# Autodesk Inventor assembly: MotorAndLoadCellBase
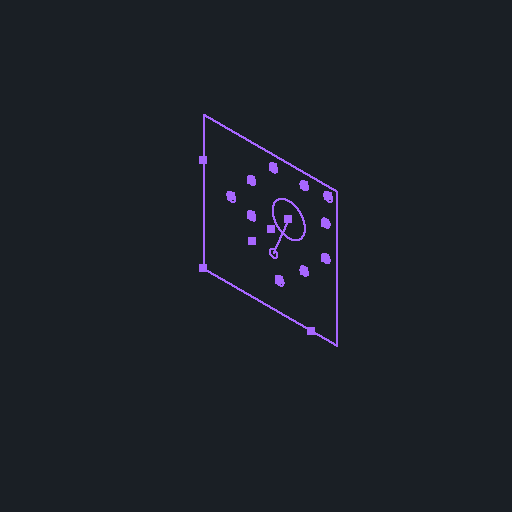
[picture p0: Inventor's stored thumbnail of the model, 512x512]
Saved by Autodesk Inventor 2024 (Build 280153000, 153)
## iProperties
Created: 2025-02-12
Part Number: MotorAndLoadCellBase
Document SubType Name: Assembly
Designer: Tommy Rohmann
Author: Tommy Rohmann
## Documents named in this file (5)
- C:\Users\Tommy Rohmann\OneDrive\Projects\Microgravity-Press-Washing-Machine\System Design and Documentation\Inventor Design Project\MotorAndLoadCellBase.iam
- C:\Users\Tommy Rohmann\OneDrive\Projects\Microgravity-Press-Washing-Machine\System Design and Documentation\Inventor Design Project\MotorAndLoadCellBase_Layout.ipt
- C:\Users\Tommy Rohmann\OneDrive\Projects\Microgravity-Press-Washing-Machine\System Design and Documentation\Inventor Design Project\StructuralBaseGuide.ipt
- C:\Users\Tommy Rohmann\OneDrive\Projects\Microgravity-Press-Washing-Machine\System Design and Documentation\Inventor Design Project\FrameGuide.ipt
- C:\Users\Tommy Rohmann\OneDrive\Projects\Microgravity-Press-Washing-Machine\System Design and Documentation\Inventor Design Project\LoadCellFootprint.ipt
## Components (4 placed, 4 different names)
1. MotorAndLoadCellBase_Layout:1
2. StructuralBaseGuide:1
3. FrameGuide:1
4. LoadCellFootprint:1
## Relationships (3: Composite 3)
- [Composite]: MotorAndLoadCellBase_Layout:1 ↔ StructuralBaseGuide:1
- [Composite]: MotorAndLoadCellBase_Layout:1 ↔ FrameGuide:1
- [Composite]: MotorAndLoadCellBase_Layout:1 ↔ LoadCellFootprint:1
